# Autodesk Inventor assembly: Test Box
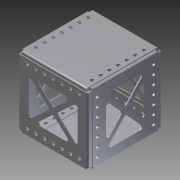
[picture p0: Inventor's stored thumbnail of the model, 180x180]
Saved by Autodesk Inventor 2012 (Build 160160000, 160)
## iProperties
Created: 2011-09-24
Part Number: Test Box
Document SubType Name: Assembly
Designer: Ian Walters
Author: Ian Walters
## Documents named in this file (3)
- C:\Users\Ian Walters\Dropbox\CAD Inventor\Preseason Projects\Test Box.iam
- C:\Users\Ian Walters\Dropbox\CAD Inventor\Preseason Projects\Test Sheet.ipt
- C:\Users\Ian Walters\Dropbox\CAD Inventor\Preseason Projects\Test Sheet 2.ipt
## Components (6 placed, 2 different names)
1. Test Sheet:1 — Insert:1, Mate:3, Insert:6, Mate:4
2. Test Sheet:2 — Insert:7, Mate:5
3. Test Sheet:3 — Insert:4, Mate:1, Insert:6, Insert:7, Mate:4, Mate:5
4. Test Sheet:4 — Insert:1, Mate:2, Insert:5, Mate:3
5. Test Sheet 2:1 — Insert:4, Mate:1
6. Test Sheet 2:2 — Mate:2, Insert:5
## Relationships (10: Insert 5, Mate 5)
- Insert:1: Test Sheet:1 ↔ Test Sheet:4
- Insert:4: Test Sheet:3 ↔ Test Sheet 2:1
- Mate:1: Test Sheet:3 ↔ Test Sheet 2:1
- Mate:2: Test Sheet:4 ↔ Test Sheet 2:2
- Insert:5: Test Sheet:4 ↔ Test Sheet 2:2
- Mate:3: Test Sheet:1 ↔ Test Sheet:4
- Insert:6: Test Sheet:1 ↔ Test Sheet:3
- Insert:7: Test Sheet:2 ↔ Test Sheet:3
- Mate:4: Test Sheet:1 ↔ Test Sheet:3
- Mate:5: Test Sheet:2 ↔ Test Sheet:3
